# Autodesk Inventor assembly: torchArm
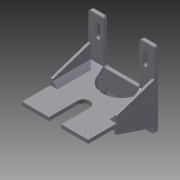
[picture p0: Inventor's stored thumbnail of the model, 180x180]
Saved by Autodesk Inventor 2013 (Build 170138000, 138)
## iProperties
Created: 2012-12-11
Part Number: torchArm
Document SubType Name: Weldment
Designer: istvan.burbank
Weld Material: Aluminum 6061, Welded
Author: istvan.burbank
## Documents named in this file (4)
- C:\Users\istvan.burbank\Documents\GitHub\Crown-Fire\CAD\CuttingHead\torchArm.iam
- C:\Users\istvan.burbank\Documents\GitHub\Crown-Fire\CAD\CuttingHead\torchArm.ipt
- C:\Users\istvan.burbank\Documents\GitHub\Crown-Fire\CAD\CuttingHead\triangleBrace.ipt
- C:\Users\istvan.burbank\Documents\GitHub\Crown-Fire\CAD\CuttingHead\torchMount_back.ipt
## Components (6 placed, 3 different names)
1. torchMount_back:1 — Mate:1, Flush:1, Mate:6, Mate:7, Mate:8, Mate:9, Flush:6
2. torchArm:1 — Mate:1, Flush:1, Mate:2, Mate:3, Mate:4, Mate:5, Flush:2, Flush:3, Flush:4, Flush:5, Flush:6
3. triangleBrace:1 — Mate:3, Flush:5, Mate:6
4. triangleBrace:2 — Mate:2, Flush:3, Mate:9
5. triangleBrace:3 — Mate:4, Flush:2, Mate:8
6. triangleBrace:4 — Mate:5, Flush:4, Mate:7
## Relationships (15: Mate 9, Flush 6)
- Mate:1: torchMount_back:1 ↔ torchArm:1
- Flush:1: torchMount_back:1 ↔ torchArm:1
- Mate:2: torchArm:1 ↔ triangleBrace:2
- Mate:3: torchArm:1 ↔ triangleBrace:1
- Mate:4: torchArm:1 ↔ triangleBrace:3
- Mate:5: torchArm:1 ↔ triangleBrace:4
- Flush:2: torchArm:1 ↔ triangleBrace:3
- Flush:3: torchArm:1 ↔ triangleBrace:2
- Flush:4: torchArm:1 ↔ triangleBrace:4
- Flush:5: torchArm:1 ↔ triangleBrace:1
- Mate:6: torchMount_back:1 ↔ triangleBrace:1
- Mate:7: torchMount_back:1 ↔ triangleBrace:4
- Mate:8: torchMount_back:1 ↔ triangleBrace:3
- Mate:9: torchMount_back:1 ↔ triangleBrace:2
- Flush:6 (5.969 mm): torchMount_back:1 ↔ torchArm:1
